# Autodesk Inventor assembly: 217-2000
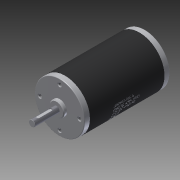
[picture p0: Inventor's stored thumbnail of the model, 180x180]
Saved by Autodesk Inventor 2015 (Build 190159000, 159)
## iProperties
Category: Motors
Company: Autodesk, Inc.
Shininess: 64.0
Length Units: 11272
Angle Units: 11279
Time Units: 11290
Mass Units: 11286
Length Display Precision: 3
Angle Display Precision: 2
Compacted: True
Document SubType Name: Assembly
Created: 2013-12-21
Project: FIRST
Part Number: 217-2000
Description: CIM Motor
Catalog Web Link: http://www.andymark.com/product-p/am-0255.htm
Vendor: AndyMark
Mass: 972.526 g
Surface Area: 376.726 cm^2
Volume: 361.438 cm^3
Density: 2.69072 g/cm^3
Density: 0.0
Volumn: 0.0
Area: 0.0
PropertySet Name: Model Information
Control State: 0
Master: False
Checked Out: False
Title: CIM Motor
Author: Autodesk, Inc.
## Documents named in this file (4)
- C:\Users\Evan\Documents\Robotics\CAD\KOP\Motors\MOT_CIM-Motor_217-2000.iam
- C:\Users\Evan\Documents\Robotics\CAD\KOP\Motors\Parts\FR801-001_CIM Motor Body.ipt
- C:\Users\Evan\Documents\Robotics\CAD\KOP\Motors\Parts\FR801-001_CIM Motor Machine Screw.ipt
- C:\Users\Evan\Documents\Robotics\CAD\KOP\Motors\MOT_CIM-Motor_217-2000_SUB.ipt
## Components (4 placed, 3 different names)
1. FR801-001_CIM Motor Body:1 — Insert:1, Insert:2
2. FR801-001_CIM Motor Machine Screw:1 — Insert:1
3. FR801-001_CIM Motor Machine Screw:2 — Insert:2
4. MOT_CIM-Motor_217-2000_SUB:1
## Relationships (2: Insert 2)
- Insert:1: FR801-001_CIM Motor Body:1 ↔ FR801-001_CIM Motor Machine Screw:1
- Insert:2: FR801-001_CIM Motor Body:1 ↔ FR801-001_CIM Motor Machine Screw:2
